# Autodesk Inventor assembly: bracketForGarageUpperAndLowerHalfs
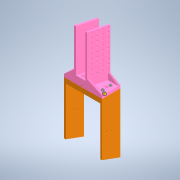
[picture p0: Inventor's stored thumbnail of the model, 180x180]
Saved by Autodesk Inventor 2022.1 (Build 261234020, 234B)
## iProperties
Created: 2021-10-28
Part Number: bracketForGarageUpperAndLowerHalfs
Document SubType Name: Assembly
Designer: robst
Author: robst
## Documents named in this file (5)
- C:\git\CAD-Development\robSteele\ShapeWays\GlobalMeteorNetwork\bracketForGarageUpperAndLowerHalfs.iam
- C:\git\CAD-Development\robSteele\ShapeWays\GlobalMeteorNetwork\bracketForGarageLowerHalf.ipt
- C:\git\CAD-Development\robSteele\ShapeWays\GlobalMeteorNetwork\bracketForGarageUpperHalf.ipt
- C:\Users\robst\Documents\Inventor\Content Center Files\R2021\en-US\ANSI B18.22.1\ANSI B18.22.1 - No. 10 - Type A.ipt
- C:\Users\robst\Documents\Inventor\Content Center Files\R2021\en-US\ANSI B18.3(11)\ANSI B18.3 - 10-32 UNF - 1.25(23).ipt
## Components (10 placed, 4 different names)
1. bracketForGarageLowerHalf:1 — Flush:2, Mate:9, Flush:3, Flush:4
2. bracketForGarageUpperHalf:1 — Flush:2, Mate:9, Flush:3, Flush:4, Mate:10, Mate:11, Mate:12, Mate:13, Mate:14, Mate:15, Mate:16, Mate:17
3. Spline Socket Button Head Cap Screw - Inch 10-32 UNF - 1.25:1 — Insert:1
4. Plain Washer (Inch) No. 10 - Type A:1 — Mate:10, Mate:11, Insert:1
5. Plain Washer (Inch) No. 10 - Type A:2 — Mate:12, Mate:13, Insert:2
6. Plain Washer (Inch) No. 10 - Type A:3 — Mate:14, Mate:15, Insert:3
7. Plain Washer (Inch) No. 10 - Type A:4 — Mate:16, Mate:17, Insert:4
8. Spline Socket Button Head Cap Screw - Inch 10-32 UNF - 1.25:2 — Insert:2
9. Spline Socket Button Head Cap Screw - Inch 10-32 UNF - 1.25:3 — Insert:3
10. Spline Socket Button Head Cap Screw - Inch 10-32 UNF - 1.25:4 — Insert:4
## Relationships (16: Mate 9, Insert 4, Flush 3)
- Flush:2: bracketForGarageLowerHalf:1 ↔ bracketForGarageUpperHalf:1
- Mate:9: bracketForGarageLowerHalf:1 ↔ bracketForGarageUpperHalf:1
- Flush:3: bracketForGarageLowerHalf:1 ↔ bracketForGarageUpperHalf:1
- Flush:4: bracketForGarageLowerHalf:1 ↔ bracketForGarageUpperHalf:1
- Mate:10: bracketForGarageUpperHalf:1 ↔ Plain Washer (Inch) No. 10 - Type A:1
- Mate:11: bracketForGarageUpperHalf:1 ↔ Plain Washer (Inch) No. 10 - Type A:1
- Mate:12: bracketForGarageUpperHalf:1 ↔ Plain Washer (Inch) No. 10 - Type A:2
- Mate:13: bracketForGarageUpperHalf:1 ↔ Plain Washer (Inch) No. 10 - Type A:2
- Mate:14: bracketForGarageUpperHalf:1 ↔ Plain Washer (Inch) No. 10 - Type A:3
- Mate:15: bracketForGarageUpperHalf:1 ↔ Plain Washer (Inch) No. 10 - Type A:3
- Mate:16: bracketForGarageUpperHalf:1 ↔ Plain Washer (Inch) No. 10 - Type A:4
- Mate:17: bracketForGarageUpperHalf:1 ↔ Plain Washer (Inch) No. 10 - Type A:4
- Insert:1: Spline Socket Button Head Cap Screw - Inch 10-32 UNF - 1.25:1 ↔ Plain Washer (Inch) No. 10 - Type A:1
- Insert:2: Plain Washer (Inch) No. 10 - Type A:2 ↔ Spline Socket Button Head Cap Screw - Inch 10-32 UNF - 1.25:2
- Insert:3: Plain Washer (Inch) No. 10 - Type A:3 ↔ Spline Socket Button Head Cap Screw - Inch 10-32 UNF - 1.25:3
- Insert:4: Plain Washer (Inch) No. 10 - Type A:4 ↔ Spline Socket Button Head Cap Screw - Inch 10-32 UNF - 1.25:4
